# Autodesk Inventor assembly: 240626_tableA
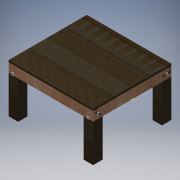
[picture p0: Inventor's stored thumbnail of the model, 180x180]
Saved by Autodesk Inventor 2016 (Build 200138000, 138)
## iProperties
Created: 2024-06-26
Part Number: 240626_tableA
Material: 일반
Document SubType Name: Assembly
Designer: pc
Author: pc
## Documents named in this file (5)
- D:\CAD_HCH\240626\240626_tableA.iam
- D:\CAD_HCH\240626\240626_tablep2.ipt
- D:\CAD_HCH\240626\240626_tablep1.ipt
- D:\CAD_HCH\240626\240626_tablep3.ipt
- C:\Users\pc\Documents\Inventor\Content Center Files\R2016\ko-KR\ANSI B18.2.3.2M(1)\ANSI B18.2.3.2M - M5x0.8 x 8(2)8.ipt
## Components (22 placed, 4 different names)
1. 240626_tablep1:1 — 메이트:1, 플러쉬:1, 플러쉬:2, 메이트:2, 플러쉬:3, 플러쉬:4, 메이트:3, 플러쉬:5, 플러쉬:6, 메이트:4, 플러쉬:7, 플러쉬:8, 메이트:5, 플러쉬:9, 플러쉬:10, 삽입:1, 삽입:2, 삽입:3, 삽입:4, 삽입:5, 삽입:6, 메이트:6, 메이트:7, 메이트:8, 메이트:9
2. 240626_tablep3:1 — 메이트:2, 플러쉬:3, 플러쉬:4
3. 240626_tablep3:2 — 메이트:3, 플러쉬:5, 플러쉬:6
4. 240626_tablep3:3 — 메이트:4, 플러쉬:7, 플러쉬:8
5. 240626_tablep3:4 — 메이트:5, 플러쉬:9, 플러쉬:10
6. 6각 나사 - 미터 (1) M5x0.8 x 8:1 — 삽입:1
7. 6각 나사 - 미터 (1) M5x0.8 x 8:2 — 삽입:2
8. 6각 나사 - 미터 (1) M5x0.8 x 8:3 — 삽입:3
9. 6각 나사 - 미터 (1) M5x0.8 x 8:4 — 삽입:4
10. 6각 나사 - 미터 (1) M5x0.8 x 8:5 — 삽입:5
11. 6각 나사 - 미터 (1) M5x0.8 x 8:6 — 삽입:6
12. 6각 나사 - 미터 (1) M5x0.8 x 8:7 — 메이트:6, 메이트:7
13. 6각 나사 - 미터 (1) M5x0.8 x 8:8 — 메이트:8, 메이트:9
14. 240626_tablep2:1 — 메이트:1, 플러쉬:1, 플러쉬:2
15. 240626_tablep2:2
16. 240626_tablep2:3
17. 240626_tablep2:4
18. 240626_tablep2:5
19. 240626_tablep2:6
20. 240626_tablep2:7
21. 240626_tablep2:8
22. 240626_tablep2:9
## Component patterns: (9 elements, first: 240626_tablep2:1)
## Relationships (25: Flush 10, Mate 9, Insert 6)
- 메이트:1 [Mate]: 240626_tablep1:1 ↔ 240626_tablep2:1
- 플러쉬:1 [Flush]: 240626_tablep1:1 ↔ 240626_tablep2:1
- 플러쉬:2 [Flush]: 240626_tablep1:1 ↔ 240626_tablep2:1
- 메이트:2 [Mate]: 240626_tablep1:1 ↔ 240626_tablep3:1
- 플러쉬:3 [Flush]: 240626_tablep1:1 ↔ 240626_tablep3:1
- 플러쉬:4 [Flush]: 240626_tablep1:1 ↔ 240626_tablep3:1
- 메이트:3 [Mate]: 240626_tablep1:1 ↔ 240626_tablep3:2
- 플러쉬:5 [Flush]: 240626_tablep1:1 ↔ 240626_tablep3:2
- 플러쉬:6 [Flush]: 240626_tablep1:1 ↔ 240626_tablep3:2
- 메이트:4 [Mate]: 240626_tablep1:1 ↔ 240626_tablep3:3
- 플러쉬:7 [Flush]: 240626_tablep1:1 ↔ 240626_tablep3:3
- 플러쉬:8 [Flush]: 240626_tablep1:1 ↔ 240626_tablep3:3
- 메이트:5 [Mate]: 240626_tablep1:1 ↔ 240626_tablep3:4
- 플러쉬:9 [Flush]: 240626_tablep1:1 ↔ 240626_tablep3:4
- 플러쉬:10 [Flush]: 240626_tablep1:1 ↔ 240626_tablep3:4
- 삽입:1 [Insert]: 240626_tablep1:1 ↔ 6각 나사 - 미터 (1) M5x0.8 x 8:1
- 삽입:2 [Insert]: 240626_tablep1:1 ↔ 6각 나사 - 미터 (1) M5x0.8 x 8:2
- 삽입:3 [Insert]: 240626_tablep1:1 ↔ 6각 나사 - 미터 (1) M5x0.8 x 8:3
- 삽입:4 [Insert]: 240626_tablep1:1 ↔ 6각 나사 - 미터 (1) M5x0.8 x 8:4
- 삽입:5 [Insert]: 240626_tablep1:1 ↔ 6각 나사 - 미터 (1) M5x0.8 x 8:5
- 삽입:6 [Insert]: 240626_tablep1:1 ↔ 6각 나사 - 미터 (1) M5x0.8 x 8:6
- 메이트:6 [Mate]: 240626_tablep1:1 ↔ 6각 나사 - 미터 (1) M5x0.8 x 8:7
- 메이트:7 [Mate]: 240626_tablep1:1 ↔ 6각 나사 - 미터 (1) M5x0.8 x 8:7
- 메이트:8 [Mate]: 240626_tablep1:1 ↔ 6각 나사 - 미터 (1) M5x0.8 x 8:8
- 메이트:9 [Mate]: 240626_tablep1:1 ↔ 6각 나사 - 미터 (1) M5x0.8 x 8:8
